# Autodesk Inventor assembly: Ensamblaje1
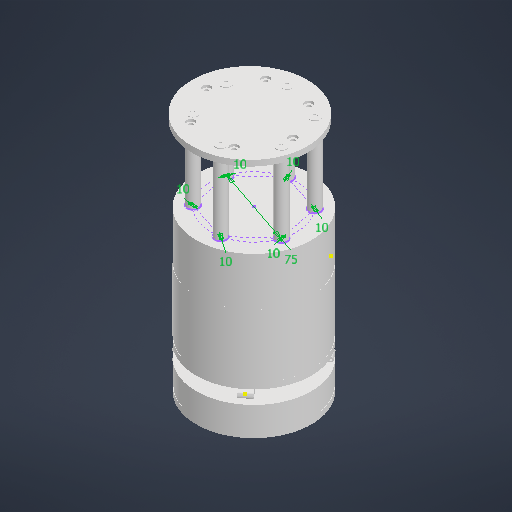
[picture p0: Inventor's stored thumbnail of the model, 512x512]
Saved by Autodesk Inventor 2026.1 (Build 301233000, 233)
## iProperties
Created: 2025-09-15
Part Number: Ensamblaje1
Document SubType Name: Assembly
Designer: Usuario
Author: Usuario
## Documents named in this file (9)
- C:\Users\vickh\Documents\Proyectos\Cansat_Huitzilin\3D\ViejoDiseno\Cansat armado.iam
- C:\Users\vickh\Documents\Proyectos\Cansat_Huitzilin\3D\ViejoDiseno\Pieza1.ipt
- C:\Users\vickh\Documents\Proyectos\Cansat_Huitzilin\3D\ViejoDiseno\Pieza2.ipt
- C:\Users\vickh\Documents\Proyectos\Cansat_Huitzilin\3D\ViejoDiseno\Pieza4.ipt
- C:\Users\vickh\Documents\Proyectos\Cansat_Huitzilin\3D\ViejoDiseno\Pieza3.ipt
- C:\Users\vickh\Documents\Proyectos\Cansat_Huitzilin\3D\ViejoDiseno\Pieza6.ipt
- C:\Users\vickh\Documents\Proyectos\Cansat_Huitzilin\3D\ViejoDiseno\Pieza5.ipt
- C:\Users\vickh\Documents\Proyectos\Cansat_Huitzilin\3D\ViejoDiseno\Pieza7.ipt
- C:\Users\vickh\Documents\Proyectos\Cansat_Huitzilin\3D\ViejoDiseno\Pieza8.ipt
## Components (8 placed, 8 different names)
1. Pieza1:1 — Insertar:1
2. Pieza2:1 — Insertar:1, Insertar:2
3. Pieza4:1 — Insertar:5
4. Pieza3:1 — Insertar:2
5. Pieza6:1
6. Pieza5:1 — Insertar:5, Insertar:6
7. Pieza7:1 — Insertar:6
8. Pieza8:1
## Relationships (4: Insert 4)
- Insertar:1: Pieza1:1 ↔ Pieza2:1
- Insertar:2: Pieza2:1 ↔ Pieza3:1
- Insertar:5: Pieza4:1 ↔ Pieza5:1
- Insertar:6: Pieza5:1 ↔ Pieza7:1
